# Autodesk Inventor assembly: Compound Layer
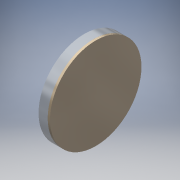
[picture p0: Inventor's stored thumbnail of the model, 180x180]
Saved by Autodesk Inventor 2017 (Build 210142000, 142)
## iProperties
Created: 2017-02-26
Part Number: Compound Layer
Document SubType Name: Assembly
Designer: Jake
Author: Jake
## Documents named in this file (3)
- C:\Users\Jake\Documents\5thYear\Project\CAD\Compound Layer.iam
- C:\Users\Jake\Documents\5thYear\Project\CAD\Vinyltoluene.ipt
- C:\Users\Jake\Documents\5thYear\Project\CAD\CD2.ipt
## Components (2 placed, 2 different names)
1. Vinyltoluene:1 — Mate:1, Mate:2
2. CD2:1 — Mate:1, Mate:2
## Relationships (2: Mate 2)
- Mate:1: Vinyltoluene:1 ↔ CD2:1
- Mate:2: Vinyltoluene:1 ↔ CD2:1
